# Autodesk Inventor assembly: WHEEL_BASE
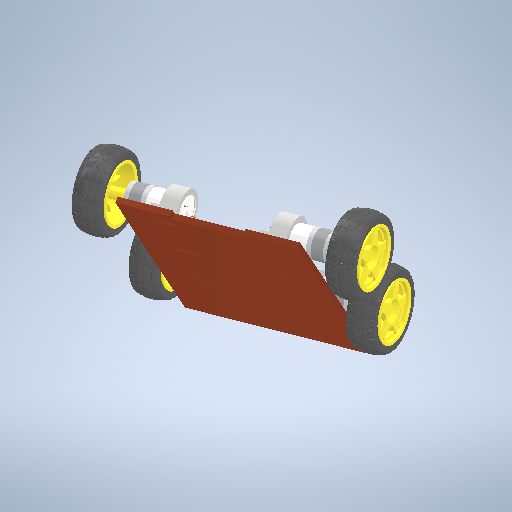
[picture p0: Inventor's stored thumbnail of the model, 512x512]
Saved by Autodesk Inventor 2025.3 (Build 293356030, 356C)
## iProperties
Created: 2026-06-30
Part Number: WHEEL_BASE
Document SubType Name: Assembly
Designer: user
Author: user
## Documents named in this file (3)
- C:\Docs\shcool\dojo\Design_3\Smaller\WHEEL_BASE.iam
- C:\Docs\shcool\dojo\Design_3\Smaller\base_2.ipt
- C:\Docs\shcool\dojo\Design_3\Smaller\motor_wheel_3.iam
## Components (5 placed, 2 different names)
1. base_2:1 — Mate:1, Mate:2, Mate:3, Mate:4, Mate:5, Mate:6, Mate:7, Mate:8, Mate:9, Mate:10, Mate:11, Mate:12
2. motor_wheel_3:1 [sub-assembly] — Mate:1, Mate:2, Mate:3
3. motor_wheel_3:2 [sub-assembly] — Mate:4, Mate:5, Mate:11
4. motor_wheel_3:3 [sub-assembly] — Mate:6, Mate:7, Mate:12
5. motor_wheel_3:4 [sub-assembly] — Mate:8, Mate:9, Mate:10
## Relationships (12: Mate 12)
- Mate:1: base_2:1 ↔ motor_wheel_3:1
- Mate:2: base_2:1 ↔ motor_wheel_3:1
- Mate:3: base_2:1 ↔ motor_wheel_3:1
- Mate:4: base_2:1 ↔ motor_wheel_3:2
- Mate:5: base_2:1 ↔ motor_wheel_3:2
- Mate:6: base_2:1 ↔ motor_wheel_3:3
- Mate:7: base_2:1 ↔ motor_wheel_3:3
- Mate:8: base_2:1 ↔ motor_wheel_3:4
- Mate:9: base_2:1 ↔ motor_wheel_3:4
- Mate:10: base_2:1 ↔ motor_wheel_3:4
- Mate:11: base_2:1 ↔ motor_wheel_3:2
- Mate:12: base_2:1 ↔ motor_wheel_3:3
